# Autodesk Inventor assembly: FrameAssembly(Printing)
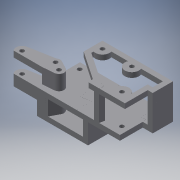
[picture p0: Inventor's stored thumbnail of the model, 180x180]
Saved by Autodesk Inventor 2017 (Build 210142000, 142)
## iProperties
Created: 2019-03-10
Part Number: FrameAssembly(Printing)
Document SubType Name: Assembly
Designer: Ben
Author: Ben
## Documents named in this file (9)
- D:\Documents\Hand Assembly V1\FrameAssembly(Printing).iam
- D:\Documents\Hand Assembly V1\Dovetail1.ipt
- D:\Documents\Hand Assembly V1\Frame VG01-04.ipt
- D:\Documents\Hand Assembly V1\Frame VG01-06.ipt
- D:\Documents\Hand Assembly V1\Frame VG01-05.ipt
- D:\Documents\Hand Assembly V1\Frame VG01-07.ipt
- D:\Documents\Hand Assembly V1\Frame VG01-1.ipt
- D:\Documents\Hand Assembly V1\Frame VG01-2.ipt
- D:\Documents\Hand Assembly V1\Frame VG01-08.ipt
## Components (8 placed, 8 different names)
1. Dovetail1:1 — Flush:16, Flush:17, Mate:14
2. Frame VG01-04:1 — Mate:6, Flush:4, Flush:5, Flush:8, Mate:7, Flush:11, Flush:12, Flush:13, Mate:9, Flush:16, Flush:17, Mate:14
3. Frame VG01-06:1 — Mate:6, Flush:4, Flush:5, Flush:9, Mate:8, Mate:11, Mate:12, Mate:13
4. Frame VG01-05:1 — Flush:8, Mate:7, Flush:10, Flush:11
5. Frame VG01-07:1 — Flush:9, Mate:8, Flush:10
6. Frame VG01-1:1 — Mate:10, Flush:14, Flush:15
7. Frame VG01-2:1 — Flush:12, Flush:13, Mate:9, Mate:10, Flush:14, Flush:15
8. Frame VG01-08:1 — Mate:11, Mate:12, Mate:13
## Relationships (21: Flush 12, Mate 9)
- Mate:6: Frame VG01-04:1 ↔ Frame VG01-06:1
- Flush:4: Frame VG01-04:1 ↔ Frame VG01-06:1
- Flush:5: Frame VG01-04:1 ↔ Frame VG01-06:1
- Flush:8: Frame VG01-04:1 ↔ Frame VG01-05:1
- Mate:7: Frame VG01-04:1 ↔ Frame VG01-05:1
- Flush:9: Frame VG01-06:1 ↔ Frame VG01-07:1
- Mate:8: Frame VG01-06:1 ↔ Frame VG01-07:1
- Flush:10: Frame VG01-05:1 ↔ Frame VG01-07:1
- Flush:11: Frame VG01-04:1 ↔ Frame VG01-05:1
- Flush:12: Frame VG01-04:1 ↔ Frame VG01-2:1
- Flush:13: Frame VG01-04:1 ↔ Frame VG01-2:1
- Mate:9: Frame VG01-04:1 ↔ Frame VG01-2:1
- Mate:10: Frame VG01-1:1 ↔ Frame VG01-2:1
- Flush:14: Frame VG01-1:1 ↔ Frame VG01-2:1
- Flush:15: Frame VG01-1:1 ↔ Frame VG01-2:1
- Mate:11: Frame VG01-06:1 ↔ Frame VG01-08:1
- Mate:12: Frame VG01-06:1 ↔ Frame VG01-08:1
- Mate:13: Frame VG01-06:1 ↔ Frame VG01-08:1
- Flush:16: Dovetail1:1 ↔ Frame VG01-04:1
- Flush:17: Dovetail1:1 ↔ Frame VG01-04:1
- Mate:14: Dovetail1:1 ↔ Frame VG01-04:1
